# Autodesk Inventor assembly: MotorBlockFirst
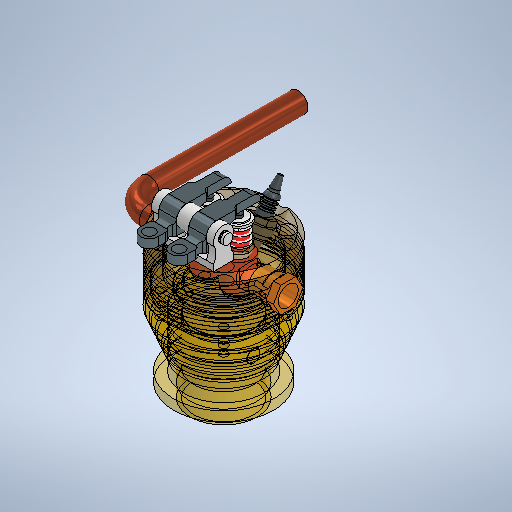
[picture p0: Inventor's stored thumbnail of the model, 512x512]
Saved by Autodesk Inventor 2025 (Build 290162010, 162A)
## iProperties
Created: 2024-07-16
Part Number: MotorBlockFirst
Document SubType Name: Assembly
Designer: ffogue
Author: ffogue
## Documents named in this file (18)
- C:\Users\Fabri\Documents\Inventor\Stermotor\MotorBlockFirst.iam
- C:\Users\Fabri\Documents\Inventor\Stermotor\Kolben.ipt
- C:\Users\Fabri\Documents\Inventor\Stermotor\KolbenFitting.ipt
- C:\Users\Fabri\Documents\Inventor\Stermotor\Ventil.ipt
- C:\Users\Fabri\Documents\Inventor\Stermotor\KopmressionsFeder_ventil.ipt
- C:\Users\Fabri\Documents\Inventor\Stermotor\ventiltasse.ipt
- C:\Users\Fabri\Documents\Inventor\Stermotor\deckeGehaeuse.ipt
- C:\Users\Fabri\Documents\Inventor\Stermotor\kipphebellagerbock.ipt
- C:\Users\Fabri\Documents\Inventor\Stermotor\Kipphebelachse.ipt
- C:\Users\Fabri\Documents\Inventor\Stermotor\KippHebel.ipt
- C:\Users\Fabri\Documents\Inventor\Stermotor\distanzbüchse_kipphebel.ipt
- C:\Users\Fabri\Documents\Inventor\Stermotor\überwurfmutter.ipt
- C:\Users\Fabri\Documents\Inventor\Stermotor\Auspuffkrümmer.ipt
- C:\Users\Fabri\Documents\Inventor\Stermotor\zündkerze.ipt
- C:\Users\Fabri\Documents\Inventor\Stermotor\gehaeuse.ipt
- C:\Users\Fabri\Documents\Inventor\Stermotor\gehaeuse2.ipt
- C:\Users\Fabri\Documents\Inventor\Stermotor\kolbenring.ipt
- C:\Users\Fabri\Documents\Inventor\Stermotor\Miederhalter_ventilfeder.ipt
## Components (23 placed, 17 different names)
1. Kolben:1 — Mate:2, Cylindrical:1, Kolbenring, Cylindrical:4, Mate:27
2. KolbenFitting:1 — Mate:2, Cylindrical:1
3. Ventil:2 — Mate:6, Insert:18, Insert:37
4. Compress Spring1:2 — Mate:8, Cylindrical:2
5. ventiltasse:1 — Mate:4, Insert:17, Mate:6, Insert:18, Mate:8, Cylindrical:2
6. ventiltasse:2 — Mate:3, Insert:16, Mate:7, Insert:19, Mate:9, Cylindrical:3, Angle:3, Mate:19, Insert:29
7. deckeGehaeuse:1 — Mate:3, Mate:4, Insert:16, Insert:17, Mate:10, Mate:11, Insert:22, Angle:1, Angle:2, Mate:16, Mate:17, Insert:27, Insert:28, Mate:18, Flush:1, Mate:21, Insert:30, Mate:28, Mate:29, Mate:30
8. Ventil:3 — Mate:7, Insert:19, Insert:36
9. Compress Spring1:3 — Mate:9, Cylindrical:3
10. kipphebellagerbock:1 — Mate:10, Mate:11, Insert:22, Mate:12, Insert:23, Insert:24
11. Kipphebelachse:1 — Mate:12, Insert:23, Mate:13, Mate:14, Mate:15
12. KippHebel:1 — Mate:13, Insert:24, Insert:25, Angle:1
13. KippHebel:2 — Mate:15, Insert:26, Angle:2
14. distanzbüchse_kipphebel:1 — Mate:14, Insert:25, Insert:26
15. überwurfmutter:2 — Mate:16, Insert:28
16. überwurfmutter:3 — Mate:17, Insert:27
17. Auspuffkrümmer:1 — Mate:20, Insert:29
18. zündkerze:1 — Mate:21, Insert:30
19. gehaeuse:1 — Mate:24, Mate:26, Mate:28, Mate:29, Insert:35
20. gehaeuse2:1 — Mate:24, Cylindrical:4, Mate:26, Mate:27, Insert:35, Mate:30
21. kolbenring:1 — Kolbenring
22. Miederhalter_ventilfeder:1 — Insert:36
23. Miederhalter_ventilfeder:2 — Insert:37
## Relationships (50: Mate 25, Insert 17, CylindricalJoint 4, Angle 3, Flush 1)
- Mate:2: Kolben:1 ↔ KolbenFitting:1
- Cylindrical:1: Kolben:1 ↔ KolbenFitting:1
- Mate:3: ventiltasse:2 ↔ deckeGehaeuse:1
- Mate:4: ventiltasse:1 ↔ deckeGehaeuse:1
- Insert:16: ventiltasse:2 ↔ deckeGehaeuse:1
- Insert:17: ventiltasse:1 ↔ deckeGehaeuse:1
- Mate:6: Ventil:2 ↔ ventiltasse:1
- Insert:18 (-2 mm): Ventil:2 ↔ ventiltasse:1
- Mate:7: ventiltasse:2 ↔ Ventil:3
- Insert:19 (-2 mm): ventiltasse:2 ↔ Ventil:3
- Mate:8: Compress Spring1:2 ↔ ventiltasse:1
- Mate:9: ventiltasse:2 ↔ Compress Spring1:3
- Cylindrical:2: Compress Spring1:2 ↔ ventiltasse:1
- Cylindrical:3: ventiltasse:2 ↔ Compress Spring1:3
- Mate:10: deckeGehaeuse:1 ↔ kipphebellagerbock:1
- Mate:11: deckeGehaeuse:1 ↔ kipphebellagerbock:1
- Insert:22: deckeGehaeuse:1 ↔ kipphebellagerbock:1
- Mate:12: kipphebellagerbock:1 ↔ Kipphebelachse:1
- Insert:23 (-26.5 mm): kipphebellagerbock:1 ↔ Kipphebelachse:1
- Mate:13: Kipphebelachse:1 ↔ KippHebel:1
- Insert:24: kipphebellagerbock:1 ↔ KippHebel:1
- Mate:14: Kipphebelachse:1 ↔ distanzbüchse_kipphebel:1
- Insert:25: KippHebel:1 ↔ distanzbüchse_kipphebel:1
- Mate:15: Kipphebelachse:1 ↔ KippHebel:2
- Insert:26: KippHebel:2 ↔ distanzbüchse_kipphebel:1
- Angle:1 (180 deg): deckeGehaeuse:1 ↔ KippHebel:1
- Angle:2 (180 deg): deckeGehaeuse:1 ↔ KippHebel:2
- Mate:16: deckeGehaeuse:1 ↔ überwurfmutter:2
- Mate:17: deckeGehaeuse:1 ↔ überwurfmutter:3
- Insert:27 (3 mm): deckeGehaeuse:1 ↔ überwurfmutter:3
- Insert:28 (3 mm): deckeGehaeuse:1 ↔ überwurfmutter:2
- Mate:18: deckeGehaeuse:1
- Flush:1: deckeGehaeuse:1
- Angle:3 (90 deg): ventiltasse:2
- Mate:19: ventiltasse:2
- Mate:20: Auspuffkrümmer:1
- Insert:29: ventiltasse:2 ↔ Auspuffkrümmer:1
- Mate:21: deckeGehaeuse:1 ↔ zündkerze:1
- Insert:30: deckeGehaeuse:1 ↔ zündkerze:1
- Mate:24: gehaeuse:1 ↔ gehaeuse2:1
- Kolbenring [Insert]: Kolben:1 ↔ kolbenring:1
- Cylindrical:4: Kolben:1 ↔ gehaeuse2:1
- Mate:26: gehaeuse:1 ↔ gehaeuse2:1
- Mate:27: Kolben:1 ↔ gehaeuse2:1
- Mate:28: deckeGehaeuse:1 ↔ gehaeuse:1
- Mate:29: deckeGehaeuse:1 ↔ gehaeuse:1
- Insert:35: gehaeuse:1 ↔ gehaeuse2:1
- Mate:30: deckeGehaeuse:1 ↔ gehaeuse2:1
- Insert:36: Ventil:3 ↔ Miederhalter_ventilfeder:1
- Insert:37: Ventil:2 ↔ Miederhalter_ventilfeder:2
